# Autodesk Inventor assembly: Assembly
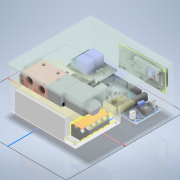
[picture p0: Inventor's stored thumbnail of the model, 180x180]
Saved by Autodesk Inventor 2022.2 (Build 262287000, 287)
## iProperties
Created: 2022-01-15
Part Number: Assembly
Document SubType Name: Assembly
Designer: siwat
Author: siwat
## Documents named in this file (11)
- D:\Git\osu-cbt\CAD\Assembly.iam
- D:\Git\osu-cbt\CAD\LM2596 DC to DC Buck Converter 3 A.ipt
- D:\Git\osu-cbt\CAD\due\ARDUINO DUE.iam
- D:\Git\osu-cbt\CAD\3V210-08NC, 2 POSITION, 3 WAY SOLENOID VALVE\3V210-08NC, 2 POSITION, 3 WAY SOLENOID VALVE.iam
- D:\Git\osu-cbt\CAD\S-60-12.ipt
- D:\Git\osu-cbt\CAD\Base.ipt
- D:\Git\osu-cbt\CAD\RelayTray.ipt
- D:\Git\osu-cbt\CAD\CoverPSU.ipt
- D:\Git\osu-cbt\CAD\2PH63091A Parts\Relay - 2 Channel - 2PH63091A - Montaj.iam
- D:\Git\osu-cbt\CAD\lcd-16x2-with-i2c-pcf8574-module-1.snapshot.2\LCD.iam
- D:\Git\osu-cbt\CAD\Lid.ipt
## Components (10 placed, 10 different names)
1. LM2596 DC to DC Buck Converter 3 A:1
2. ARDUINO DUE:1 [sub-assembly]
3. 3V210-08NC, 2 POSITION, 3 WAY SOLENOID VALVE:1 [sub-assembly]
4. S-60-12:1
5. Base:1 — Flush:1, Flush:2, Flush:3, Flush:4, Flush:5, Flush:6
6. RelayTray:1 — Flush:1, Flush:2
7. CoverPSU:1 — Flush:3, Flush:4
8. Relay - 2 Channel - 2PH63091A - Montaj:1 [sub-assembly]
9. LCD:1 [sub-assembly]
10. Lid:1 — Flush:5, Flush:6
## Relationships (6: Flush 6)
- Flush:1: Base:1 ↔ RelayTray:1
- Flush:2: Base:1 ↔ RelayTray:1
- Flush:3: Base:1 ↔ CoverPSU:1
- Flush:4: Base:1 ↔ CoverPSU:1
- Flush:5: Base:1 ↔ Lid:1
- Flush:6: Base:1 ↔ Lid:1
